# Autodesk Inventor assembly: DT Side Assembly
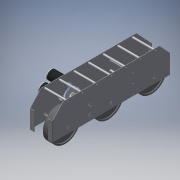
[picture p0: Inventor's stored thumbnail of the model, 180x180]
Saved by Autodesk Inventor 2016 (Build 200138000, 138)
## iProperties
Created: 2018-05-03
Part Number: DT Side Assembly
Document SubType Name: Assembly
Designer: 2000083068
Mass: 2864.4 g
Surface Area: 10801.9 cm^2
Volume: 2767.29 cm^3
Density: 1.03509 g/cm^3
Author: 2000083068
## Documents named in this file (13)
- F:\Robotics\Off Season\Blannon\DT Side Assembly.iam
- F:\Robotics\Off Season\Blannon\Fixed Side frame.ipt
- F:\Robotics\Off Season\Blannon\.5 ID Flanged Bearing.ipt
- F:\Robotics\Off Season\Blannon\ThunderHex_Stock_18in.ipt
- F:\Robotics\Off Season\Blannon\72t_Aluminum_Spur_Gear_20_DP_1_2_Hex_Bore_217-3576.ipt
- F:\Robotics\Off Season\Blannon\24t_Steel_Spur_Gear_20_DP_1_2_Hex_Bore_217-5464.ipt
- F:\Robotics\Off Season\Blannon\Cim Motor.ipt
- F:\Robotics\Off Season\Blannon\Wheel Hub.ipt
- F:\Robotics\Off Season\Blannon\30t_x_9mm_Wide_Double_Flange_Aluminum_Pulley_HTD_5mm_1_2_Hex_Bore_217-3229.ipt
- F:\Robotics\Off Season\Blannon\30t_x_15mm_Wide_Aluminum_Pulley_HTD_5mm_1_2_Hex_217-4102.ipt
- F:\Robotics\Off Season\Blannon\Fixed Side Frame Outside.ipt
- F:\Robotics\Off Season\Blannon\Delrin Spacer.ipt
- F:\Robotics\Off Season\Blannon\14t_Steel_Spur_Gear_20.ipt
## Components (44 placed, 12 different names)
1. Fixed Side frame:1 — Mate:1, Mate:2, Mate:3, Mate:20, Mate:21, Mate:23, Mate:25, Mate:39, Insert:1, Insert:2, Insert:3, Insert:4, Insert:5, Insert:6, Insert:7, Insert:8, Mate:68, Mate:69, Mate:70, Mate:76, Mate:77, Mate:78, Mate:79, Mate:80, Mate:81, Insert:15, Insert:16, Insert:17, Insert:18, Insert:19, Mate:88, Mate:89, Insert:25, Insert:26, Insert:27, Insert:28, Insert:29, Insert:30, Insert:31, Insert:32, Insert:33, Insert:34, Flush:29, Flush:30
2. 72t_Aluminum_Spur_Gear_20_DP_1_2_Hex_Bore_217-3576:1 — Insert:14, Mate:71
3. 72t_Aluminum_Spur_Gear_20_DP_1_2_Hex_Bore_217-3576:2 — Mate:74, Mate:75, Flush:19, Mate:94
4. 24t_Steel_Spur_Gear_20_DP_1_2_Hex_Bore_217-5464:1 — Mate:71, Mate:72, Mate:73, Flush:19
5. Cim Motor:1 — Mate:21, Mate:25, Insert:1, Insert:17, Insert:36
6. Cim Motor:2 — Insert:2, Insert:18, Insert:35
7. Cim Motor:3 — Mate:20, Mate:23, Insert:3, Insert:19, Insert:37
8. .5 ID Flanged Bearing:1 — Insert:4, Insert:9, Mate:80, Mate:81
9. .5 ID Flanged Bearing:2 — Insert:5, Insert:12, Mate:76, Mate:77
10. .5 ID Flanged Bearing:3 — Insert:6, Insert:10, Insert:15
11. .5 ID Flanged Bearing:4 — Insert:7, Insert:11, Insert:16
12. .5 ID Flanged Bearing:5 — Insert:8, Insert:13, Mate:78, Mate:79
13. ThunderHex_Stock_18in:1 — Insert:10, Mate:74, Mate:75, Mate:90, Mate:91
14. ThunderHex_Stock_18in:2 — Insert:11, Insert:14, Mate:72, Mate:73
15. ThunderHex_Stock_18in:3 — Insert:13, Mate:86, Mate:87, Mate:100, Mate:101
16. ThunderHex_Stock_18in:4 — Insert:9, Mate:82, Mate:83, Mate:98, Mate:99
17. ThunderHex_Stock_18in:5 — Insert:12, Mate:84, Mate:85, Mate:92, Mate:93, Mate:95, Mate:96
18. Wheel Hub:1 — Mate:82, Mate:83, Mate:102, Flush:26, Flush:27
19. Wheel Hub:3 — Mate:84, Mate:85, Flush:26
20. Wheel Hub:4 — Mate:86, Mate:87, Flush:27
21. 30t_x_9mm_Wide_Double_Flange_Aluminum_Pulley_HTD_5mm_1_2_Hex_Bore_217-3229:1 — Mate:98, Mate:99, Flush:21, Mate:102
22. 30t_x_9mm_Wide_Double_Flange_Aluminum_Pulley_HTD_5mm_1_2_Hex_Bore_217-3229:2 — Flush:22, Mate:100, Mate:101
23. 30t_x_9mm_Wide_Double_Flange_Aluminum_Pulley_HTD_5mm_1_2_Hex_Bore_217-3229:3 — Mate:90, Mate:91, Mate:94, Flush:20
24. 30t_x_9mm_Wide_Double_Flange_Aluminum_Pulley_HTD_5mm_1_2_Hex_Bore_217-3229:4 — Mate:92, Mate:93, Flush:20, Mate:97
25. 30t_x_15mm_Wide_Aluminum_Pulley_HTD_5mm_1_2_Hex_217-4102:1 — Mate:95, Mate:96, Mate:97, Flush:21, Flush:22
26. Fixed Side Frame Outside:1 — Flush:29, Flush:30
27. .5 ID Flanged Bearing:6
28. .5 ID Flanged Bearing:7
29. .5 ID Flanged Bearing:8
30. .5 ID Flanged Bearing:9
31. .5 ID Flanged Bearing:10
32. Delrin Spacer:1 — Insert:34
33. Delrin Spacer:2 — Insert:33
34. Delrin Spacer:3 — Insert:32
35. Delrin Spacer:4 — Insert:31
36. Delrin Spacer:5 — Insert:30
37. Delrin Spacer:6 — Insert:29
38. Delrin Spacer:7 — Insert:28
39. Delrin Spacer:8 — Insert:27
40. Delrin Spacer:9 — Insert:26
41. Delrin Spacer:10 — Insert:25
42. 14t_Steel_Spur_Gear_20:1 — Insert:35
43. 14t_Steel_Spur_Gear_20:2 — Insert:36
44. 14t_Steel_Spur_Gear_20:3 — Insert:37
## Relationships (83: Mate 43, Insert 32, Flush 8)
- Mate:1: Fixed Side frame:1
- Mate:2 (127 mm): Fixed Side frame:1
- Mate:3: Fixed Side frame:1
- Mate:20: Fixed Side frame:1 ↔ Cim Motor:3
- Mate:21: Fixed Side frame:1 ↔ Cim Motor:1
- Mate:23: Fixed Side frame:1 ↔ Cim Motor:3
- Mate:25: Fixed Side frame:1 ↔ Cim Motor:1
- Mate:39: Fixed Side frame:1
- Insert:1: Fixed Side frame:1 ↔ Cim Motor:1
- Insert:2: Fixed Side frame:1 ↔ Cim Motor:2
- Insert:3: Fixed Side frame:1 ↔ Cim Motor:3
- Insert:4: Fixed Side frame:1 ↔ .5 ID Flanged Bearing:1
- Insert:5: Fixed Side frame:1 ↔ .5 ID Flanged Bearing:2
- Insert:6: Fixed Side frame:1 ↔ .5 ID Flanged Bearing:3
- Insert:7: Fixed Side frame:1 ↔ .5 ID Flanged Bearing:4
- Insert:8: Fixed Side frame:1 ↔ .5 ID Flanged Bearing:5
- Insert:9: .5 ID Flanged Bearing:1 ↔ ThunderHex_Stock_18in:4
- Insert:10: .5 ID Flanged Bearing:3 ↔ ThunderHex_Stock_18in:1
- Insert:11: .5 ID Flanged Bearing:4 ↔ ThunderHex_Stock_18in:2
- Insert:12 (6.35 mm): .5 ID Flanged Bearing:2 ↔ ThunderHex_Stock_18in:5
- Insert:13: .5 ID Flanged Bearing:5 ↔ ThunderHex_Stock_18in:3
- Mate:68: Fixed Side frame:1
- Mate:69: Fixed Side frame:1
- Mate:70: Fixed Side frame:1
- Insert:14 (-25.4 mm): 72t_Aluminum_Spur_Gear_20_DP_1_2_Hex_Bore_217-3576:1 ↔ ThunderHex_Stock_18in:2
- Mate:71: 72t_Aluminum_Spur_Gear_20_DP_1_2_Hex_Bore_217-3576:1 ↔ 24t_Steel_Spur_Gear_20_DP_1_2_Hex_Bore_217-5464:1
- Mate:72: 24t_Steel_Spur_Gear_20_DP_1_2_Hex_Bore_217-5464:1 ↔ ThunderHex_Stock_18in:2
- Mate:73: 24t_Steel_Spur_Gear_20_DP_1_2_Hex_Bore_217-5464:1 ↔ ThunderHex_Stock_18in:2
- Mate:74: 72t_Aluminum_Spur_Gear_20_DP_1_2_Hex_Bore_217-3576:2 ↔ ThunderHex_Stock_18in:1
- Mate:75: 72t_Aluminum_Spur_Gear_20_DP_1_2_Hex_Bore_217-3576:2 ↔ ThunderHex_Stock_18in:1
- Mate:76: Fixed Side frame:1 ↔ .5 ID Flanged Bearing:2
- Mate:77: Fixed Side frame:1 ↔ .5 ID Flanged Bearing:2
- Mate:78: Fixed Side frame:1 ↔ .5 ID Flanged Bearing:5
- Mate:79: Fixed Side frame:1 ↔ .5 ID Flanged Bearing:5
- Mate:80: Fixed Side frame:1 ↔ .5 ID Flanged Bearing:1
- Mate:81: Fixed Side frame:1 ↔ .5 ID Flanged Bearing:1
- Insert:15 (-6.35 mm): Fixed Side frame:1 ↔ .5 ID Flanged Bearing:3
- Flush:19: 72t_Aluminum_Spur_Gear_20_DP_1_2_Hex_Bore_217-3576:2 ↔ 24t_Steel_Spur_Gear_20_DP_1_2_Hex_Bore_217-5464:1
- Insert:16: Fixed Side frame:1 ↔ .5 ID Flanged Bearing:4
- Insert:17 (3.175 mm): Fixed Side frame:1 ↔ Cim Motor:1
- Insert:18 (3.175 mm): Fixed Side frame:1 ↔ Cim Motor:2
- Insert:19 (3.175 mm): Fixed Side frame:1 ↔ Cim Motor:3
- Mate:82: ThunderHex_Stock_18in:4 ↔ Wheel Hub:1
- Mate:83: ThunderHex_Stock_18in:4 ↔ Wheel Hub:1
- Mate:84: ThunderHex_Stock_18in:5 ↔ Wheel Hub:3
- Mate:85: ThunderHex_Stock_18in:5 ↔ Wheel Hub:3
- Mate:86: ThunderHex_Stock_18in:3 ↔ Wheel Hub:4
- Mate:87: ThunderHex_Stock_18in:3 ↔ Wheel Hub:4
- Mate:88: Fixed Side frame:1
- Mate:89: Fixed Side frame:1
- Mate:90: ThunderHex_Stock_18in:1 ↔ 30t_x_9mm_Wide_Double_Flange_Aluminum_Pulley_HTD_5mm_1_2_Hex_Bore_217-3229:3
- Mate:91: ThunderHex_Stock_18in:1 ↔ 30t_x_9mm_Wide_Double_Flange_Aluminum_Pulley_HTD_5mm_1_2_Hex_Bore_217-3229:3
- Mate:92: ThunderHex_Stock_18in:5 ↔ 30t_x_9mm_Wide_Double_Flange_Aluminum_Pulley_HTD_5mm_1_2_Hex_Bore_217-3229:4
- Mate:93: ThunderHex_Stock_18in:5 ↔ 30t_x_9mm_Wide_Double_Flange_Aluminum_Pulley_HTD_5mm_1_2_Hex_Bore_217-3229:4
- Mate:94 (3.175 mm): 72t_Aluminum_Spur_Gear_20_DP_1_2_Hex_Bore_217-3576:2 ↔ 30t_x_9mm_Wide_Double_Flange_Aluminum_Pulley_HTD_5mm_1_2_Hex_Bore_217-3229:3
- Flush:20: 30t_x_9mm_Wide_Double_Flange_Aluminum_Pulley_HTD_5mm_1_2_Hex_Bore_217-3229:3 ↔ 30t_x_9mm_Wide_Double_Flange_Aluminum_Pulley_HTD_5mm_1_2_Hex_Bore_217-3229:4
- Mate:95: ThunderHex_Stock_18in:5 ↔ 30t_x_15mm_Wide_Aluminum_Pulley_HTD_5mm_1_2_Hex_217-4102:1
- Mate:96: ThunderHex_Stock_18in:5 ↔ 30t_x_15mm_Wide_Aluminum_Pulley_HTD_5mm_1_2_Hex_217-4102:1
- Mate:97: 30t_x_9mm_Wide_Double_Flange_Aluminum_Pulley_HTD_5mm_1_2_Hex_Bore_217-3229:4 ↔ 30t_x_15mm_Wide_Aluminum_Pulley_HTD_5mm_1_2_Hex_217-4102:1
- Mate:98: ThunderHex_Stock_18in:4 ↔ 30t_x_9mm_Wide_Double_Flange_Aluminum_Pulley_HTD_5mm_1_2_Hex_Bore_217-3229:1
- Mate:99: ThunderHex_Stock_18in:4 ↔ 30t_x_9mm_Wide_Double_Flange_Aluminum_Pulley_HTD_5mm_1_2_Hex_Bore_217-3229:1
- Flush:21: 30t_x_9mm_Wide_Double_Flange_Aluminum_Pulley_HTD_5mm_1_2_Hex_Bore_217-3229:1 ↔ 30t_x_15mm_Wide_Aluminum_Pulley_HTD_5mm_1_2_Hex_217-4102:1
- Flush:22: 30t_x_9mm_Wide_Double_Flange_Aluminum_Pulley_HTD_5mm_1_2_Hex_Bore_217-3229:2 ↔ 30t_x_15mm_Wide_Aluminum_Pulley_HTD_5mm_1_2_Hex_217-4102:1
- Mate:100: ThunderHex_Stock_18in:3 ↔ 30t_x_9mm_Wide_Double_Flange_Aluminum_Pulley_HTD_5mm_1_2_Hex_Bore_217-3229:2
- Mate:101: ThunderHex_Stock_18in:3 ↔ 30t_x_9mm_Wide_Double_Flange_Aluminum_Pulley_HTD_5mm_1_2_Hex_Bore_217-3229:2
- Mate:102 (3.175 mm): Wheel Hub:1 ↔ 30t_x_9mm_Wide_Double_Flange_Aluminum_Pulley_HTD_5mm_1_2_Hex_Bore_217-3229:1
- Flush:26: Wheel Hub:1 ↔ Wheel Hub:3
- Flush:27: Wheel Hub:1 ↔ Wheel Hub:4
- Insert:25: Fixed Side frame:1 ↔ Delrin Spacer:10
- Insert:26: Fixed Side frame:1 ↔ Delrin Spacer:9
- Insert:27: Fixed Side frame:1 ↔ Delrin Spacer:8
- Insert:28: Fixed Side frame:1 ↔ Delrin Spacer:7
- Insert:29: Fixed Side frame:1 ↔ Delrin Spacer:6
- Insert:30: Fixed Side frame:1 ↔ Delrin Spacer:5
- Insert:31: Fixed Side frame:1 ↔ Delrin Spacer:4
- Insert:32: Fixed Side frame:1 ↔ Delrin Spacer:3
- Insert:33: Fixed Side frame:1 ↔ Delrin Spacer:2
- Insert:34: Fixed Side frame:1 ↔ Delrin Spacer:1
- Flush:29: Fixed Side frame:1 ↔ Fixed Side Frame Outside:1
- Flush:30: Fixed Side frame:1 ↔ Fixed Side Frame Outside:1
- Insert:35 (6.35 mm): Cim Motor:2 ↔ 14t_Steel_Spur_Gear_20:1
- Insert:36 (6.35 mm): Cim Motor:1 ↔ 14t_Steel_Spur_Gear_20:2
- Insert:37 (6.35 mm): Cim Motor:3 ↔ 14t_Steel_Spur_Gear_20:3
